# Autodesk Inventor assembly: Montagem peças 11 a 14
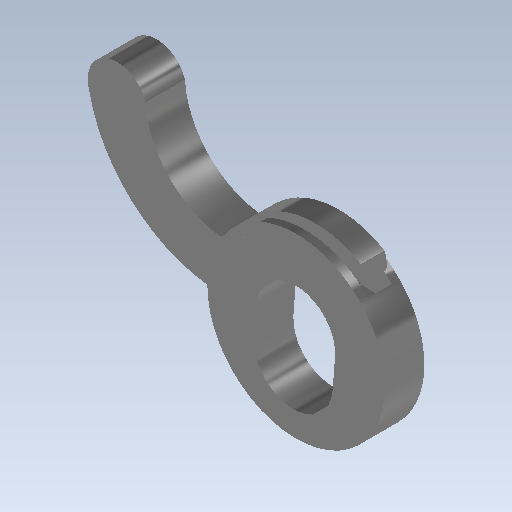
[picture p0: Inventor's stored thumbnail of the model, 512x512]
Saved by Autodesk Inventor 2021 (Build 250183000, 183)
## iProperties
Created: 2020-11-29
Part Number: Montagem peças 11 a 14
Document SubType Name: Assembly
Designer: Bruno
Author: Bruno
## Documents named in this file (5)
- C:\Users\Public\Documents\Autodesk\Inventor 2021\Montagem peças 11 a 14.iam
- C:\Users\Public\Documents\Autodesk\Inventor 2021\Peça 12.ipt
- C:\Users\Bruno\Documents\Quadirmestre Suplementar\Projeto Assistido por Computador\Peça_11.ipt
- C:\Users\Public\Documents\Autodesk\Inventor 2021\Peça 13.ipt
- C:\Users\Public\Documents\Autodesk\Inventor 2021\Peça14.ipt
## Components (4 placed, 4 different names)
1. Peça 12:1 — Coincidente:1, Rotativa:1, Coincidente:2
2. Peça_11:1 — Coincidente:1, Rotativa:1, Coincidente:3, Coincidente:4, Alinhado:1
3. Peça 13:1 — Coincidente:2, Coincidente:3
4. Peça14:1 — Coincidente:4, Alinhado:1
## Relationships (6: Mate 4, RevoluteJoint 1, Flush 1)
- Coincidente:1 [Mate]: Peça 12:1 ↔ Peça_11:1
- Rotativa:1 [RevoluteJoint]: Peça 12:1 ↔ Peça_11:1
- Coincidente:2 [Mate]: Peça 12:1 ↔ Peça 13:1
- Coincidente:3 [Mate]: Peça_11:1 ↔ Peça 13:1
- Coincidente:4 [Mate]: Peça_11:1 ↔ Peça14:1
- Alinhado:1 [Flush]: Peça_11:1 ↔ Peça14:1
